# Autodesk Inventor assembly: Mount
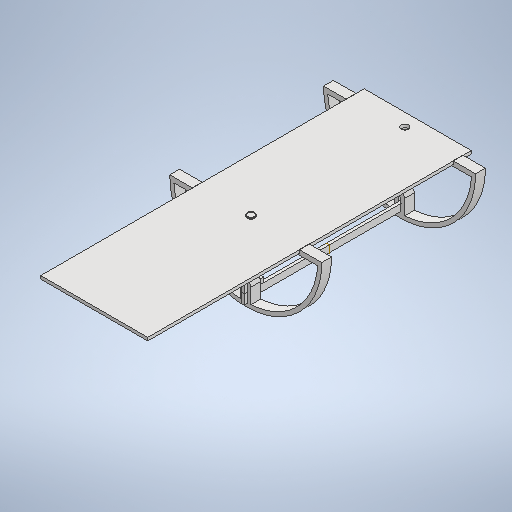
[picture p0: Inventor's stored thumbnail of the model, 512x512]
Saved by Autodesk Inventor 2025 (Build 290162010, 162A)
## iProperties
Created: 2024-06-06
Part Number: Mount
Document SubType Name: Assembly
Designer: vncnt
Author: vncnt
## Documents named in this file (7)
- C:\Users\vncnt\City Tech Dropbox\Vincent Ching\Community Sensor Lab Program\CAD\Air Quality Board Mount\Mount.iam
- C:\Users\vncnt\City Tech Dropbox\Vincent Ching\Community Sensor Lab Program\CAD\Air Quality Board Mount\Siding Lock.ipt
- C:\Users\vncnt\City Tech Dropbox\Vincent Ching\Community Sensor Lab Program\CAD\Air Quality Board Mount\Bar.ipt
- C:\Users\vncnt\City Tech Dropbox\Vincent Ching\Community Sensor Lab Program\CAD\Air Quality Board Mount\Board.ipt
- C:\Users\vncnt\City Tech Dropbox\Vincent Ching\Community Sensor Lab Program\CAD\Air Quality Board Mount\Key.ipt
- C:\Users\vncnt\City Tech Dropbox\Vincent Ching\Community Sensor Lab Program\CAD\Air Quality Board Mount\Pin Hole Lock.ipt
- C:\Users\vncnt\City Tech Dropbox\Vincent Ching\Community Sensor Lab Program\CAD\Air Quality Board Mount\Pin Hole Lock2.ipt
## Components (7 placed, 6 different names)
1. Siding Lock:1 — Mate:9, Mate:10, Mate:12
2. Siding Lock:2 — Mate:3, Mate:4, Mate:5, Mate:6, Mate:7, Mate:11, Mate:14
3. Bar:1 — Mate:4, Mate:5, Mate:6, Flush:1, Mate:8, Mate:9, Mate:10
4. Board:1 — Mate:3, Mate:11, Mate:12, Mate:13
5. Key:1 — Mate:7, Flush:1, Mate:8
6. Pin Hole Lock:1 — Mate:13
7. Pin Hole Lock2:1 — Mate:14
## Relationships (13: Mate 12, Flush 1)
- Mate:3: Siding Lock:2 ↔ Board:1
- Mate:4: Siding Lock:2 ↔ Bar:1
- Mate:5: Siding Lock:2 ↔ Bar:1
- Mate:6: Siding Lock:2 ↔ Bar:1
- Mate:7: Siding Lock:2 ↔ Key:1
- Flush:1: Bar:1 ↔ Key:1
- Mate:8: Bar:1 ↔ Key:1
- Mate:9: Siding Lock:1 ↔ Bar:1
- Mate:10: Siding Lock:1 ↔ Bar:1
- Mate:11: Siding Lock:2 ↔ Board:1
- Mate:12: Siding Lock:1 ↔ Board:1
- Mate:13: Board:1 ↔ Pin Hole Lock:1
- Mate:14: Siding Lock:2 ↔ Pin Hole Lock2:1
